# Autodesk Inventor assembly: 2段目
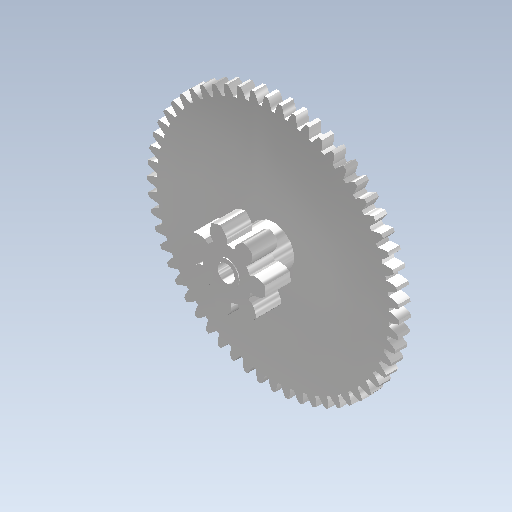
[picture p0: Inventor's stored thumbnail of the model, 512x512]
Saved by Autodesk Inventor 2020.4 (Build 244396000, 396)
## iProperties
Created: 2021-04-23
Part Number: 2段目
Document SubType Name: Assembly
Designer: happy
Mass: 23.5052 g
Surface Area: 80.0622 cm^2
Volume: 8.39472 cm^3
Density: 2.8 g/cm^3
Author: happy
## Documents named in this file (7)
- C:\Users\happy\OneDrive\ドキュメント\賢一ファイル\SRDC\試作10-2\アームギア\2段目.iam
- C:\Users\happy\OneDrive\ドキュメント\賢一ファイル\SRDC\試作10-2\アームギア\2ギア接続部.ipt
- C:\Users\happy\OneDrive\ドキュメント\賢一ファイル\SRDC\試作10-2\アームギア\2ギア接続部外.ipt
- C:\Users\happy\OneDrive\ドキュメント\賢一ファイル\SRDC\試作10-2\アームギア\m1z57.ipt
- C:\Users\happy\OneDrive\ドキュメント\賢一ファイル\SRDC\試作10-2\アームギア\m2z7.ipt
- C:\Users\happy\OneDrive\ドキュメント\賢一ファイル\SRDC\試作10-2\アームギア\2ギア接続部.m2側ipt.ipt
- C:\Users\happy\OneDrive\ドキュメント\賢一ファイル\SRDC\試作10-2\アームギア\2段目スペーサ.ipt
## Components (7 placed, 6 different names)
1. 2ギア接続部:1 — 挿入:3, 挿入:7, 挿入:8, メイト:6
2. 2ギア接続部外:1 — メイト:1, 挿入:5, メイト:4
3. m1z57:1 — 挿入:5, 挿入:7
4. m2z7:1 — 挿入:6, 挿入:9, メイト:5
5. 2ギア接続部.m2側ipt:1 — 挿入:3, メイト:1, 挿入:6, メイト:4, メイト:5, メイト:6
6. 2段目スペーサ:1 — 挿入:8
7. 2段目スペーサ:2 — 挿入:9
## Relationships (10: Insert 6, Mate 4)
- 挿入:3 [Insert]: 2ギア接続部:1 ↔ 2ギア接続部.m2側ipt:1
- メイト:1 [Mate]: 2ギア接続部外:1 ↔ 2ギア接続部.m2側ipt:1
- 挿入:5 [Insert]: 2ギア接続部外:1 ↔ m1z57:1
- 挿入:6 [Insert]: m2z7:1 ↔ 2ギア接続部.m2側ipt:1
- 挿入:7 [Insert]: 2ギア接続部:1 ↔ m1z57:1
- 挿入:8 [Insert]: 2ギア接続部:1 ↔ 2段目スペーサ:1
- 挿入:9 [Insert]: m2z7:1 ↔ 2段目スペーサ:2
- メイト:4 [Mate]: 2ギア接続部外:1 ↔ 2ギア接続部.m2側ipt:1
- メイト:5 [Mate]: m2z7:1 ↔ 2ギア接続部.m2側ipt:1
- メイト:6 [Mate]: 2ギア接続部:1 ↔ 2ギア接続部.m2側ipt:1
